# Autodesk Inventor assembly: RobotArm VersaPlanetaryGearbox
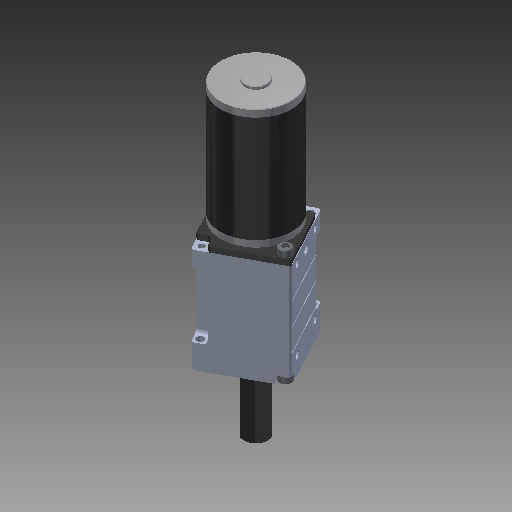
[picture p0: Inventor's stored thumbnail of the model, 512x512]
Saved by Autodesk Inventor 2018 (Build 220112000, 112)
## iProperties
Created: 2014-02-17
Part Number: RobotArm VersaPlanetaryGearbox
Description: STEP AP214
Document SubType Name: Assembly
Designer: lopez.xavier
Sending System: SolidWorks 2013
Preprocessor: SwSTEP 2.0
Title: BAG 2 stage Release.STEP
Author: IFMI-VEX04
Revision Number: ANY
## Documents named in this file (17)
- \\fs1\studentusers\class19\Lopez.Xavier\documents\RobotArm VersaPlanetaryGearbox.iam
- C:\Users\lopez.xavier.NICHOLSNT.000\Downloads\217-2625-001 Rev1.ipt
- C:\Users\lopez.xavier.NICHOLSNT.000\Downloads\217-2625-002 Rev1.ipt
- C:\Users\lopez.xavier.NICHOLSNT.000\Downloads\217-2625-003 Rev1.ipt
- C:\Users\lopez.xavier.NICHOLSNT.000\Downloads\217-2625-009 Rev1.ipt
- C:\Users\lopez.xavier.NICHOLSNT.000\Downloads\217-2625-100.iam
- C:\Users\lopez.xavier.NICHOLSNT.000\Downloads\217-2625-007 Rev1_Sun_Driver01.ipt
- C:\Users\lopez.xavier.NICHOLSNT.000\Downloads\217-2742.ipt
- C:\Users\lopez.xavier.NICHOLSNT.000\Downloads\SSS1032-0125ZB_94105A824.ipt
- C:\Users\lopez.xavier.NICHOLSNT.000\Downloads\217-3351.ipt
- C:\Users\lopez.xavier.NICHOLSNT.000\Downloads\217-2816-001 Rev1.ipt
- C:\Users\lopez.xavier.NICHOLSNT.000\Downloads\SSA_SSA0832-1750ZC.ipt
- C:\Users\lopez.xavier.NICHOLSNT.000\Downloads\217-2625-011 Rev1.ipt
- C:\Users\lopez.xavier.NICHOLSNT.000\Downloads\SSA_SSA0832-0500ZC.ipt
- C:\Users\lopez.xavier.NICHOLSNT.000\Downloads\SSHCM004_SSHCM004070010C.ipt
- C:\Users\lopez.xavier.NICHOLSNT.000\Downloads\217-2818 Rev1.iam
- C:\Users\lopez.xavier.NICHOLSNT.000\Downloads\217-2822-003 Rev4.ipt
## Components (21 placed, 21 different names)
1. 217-2625-001 Rev1_1 — Mate:41, Flush:10, Flush:11, Mate:49, Flush:13, Mate:57
2. 217-2625-002 Rev1_2 — Mate:13, Mate:15, Mate:16, Mate:17, Mate:18, Mate:19, Flush:12, Mate:50
3. 217-2625-003 Rev1_3 — Mate:11, Mate:14
4. 217-2625-009 Rev1_4 — Mate:20, Flush:9, Mate:27, Mate:47, Mate:48, Flush:13
5. 217-2625-100_5 [sub-assembly] — Mate:33, Mate:44, Mate:45
6. 217-2625-007 Rev1_Sun_Driver01_6 — Mate:47
7. 217-2742_7 — Mate:11, Mate:12, Mate:13, Mate:14, Mate:15
8. 217-2742_8 — Mate:12, Flush:12
9. SSS1032-0125ZB_94105A824_12 — Mate:27, Mate:46
10. 217-3351_14 — Mate:22, Mate:40, Mate:58
11. 217-2816-001 Rev1_15 — Mate:42, Mate:43, Mate:50, Mate:51, Mate:52
12. SSA_SSA0832-1750ZC_16 — Mate:16, Mate:17, Mate:54, Mate:56
13. SSA_SSA0832-1750ZC_17 — Mate:18, Mate:19, Mate:53, Mate:55
14. 217-2625-011 Rev1_18 — Mate:20, Flush:9, Mate:46
15. SSA_SSA0832-0500ZC_19 — Mate:37, Mate:39, Mate:55
16. SSA_SSA0832-0500ZC_20 — Mate:36, Mate:38, Mate:56
17. SSHCM004_SSHCM004070010C_21 — Mate:24, Mate:25
18. SSHCM004_SSHCM004070010C_22 — Mate:23, Mate:26, Mate:40
19. 217-2816-001 Rev1_23 — Mate:44, Mate:45, Mate:48, Mate:49, Mate:51, Mate:52, Mate:53, Mate:54, Mate:57
20. 217-2818 Rev1_24 [sub-assembly] — Mate:33, Mate:42, Mate:43
21. 217-2822-003 Rev4_25 — Mate:22, Mate:23, Mate:24, Mate:25, Mate:26, Mate:36, Mate:37, Mate:38, Mate:39, Mate:41, Flush:10, Flush:11, Mate:58
## Relationships (45: Mate 40, Flush 5)
- Mate:11: 217-2625-003 Rev1_3 ↔ 217-2742_7
- Mate:12: 217-2742_7 ↔ 217-2742_8
- Mate:13: 217-2625-002 Rev1_2 ↔ 217-2742_7
- Mate:14: 217-2625-003 Rev1_3 ↔ 217-2742_7
- Mate:15: 217-2625-002 Rev1_2 ↔ 217-2742_7
- Mate:16: 217-2625-002 Rev1_2 ↔ SSA_SSA0832-1750ZC_16
- Mate:17: 217-2625-002 Rev1_2 ↔ SSA_SSA0832-1750ZC_16
- Mate:18: 217-2625-002 Rev1_2 ↔ SSA_SSA0832-1750ZC_17
- Mate:19: 217-2625-002 Rev1_2 ↔ SSA_SSA0832-1750ZC_17
- Mate:20: 217-2625-009 Rev1_4 ↔ 217-2625-011 Rev1_18
- Flush:9: 217-2625-009 Rev1_4 ↔ 217-2625-011 Rev1_18
- Mate:22: 217-3351_14 ↔ 217-2822-003 Rev4_25
- Mate:23: SSHCM004_SSHCM004070010C_22 ↔ 217-2822-003 Rev4_25
- Mate:24: SSHCM004_SSHCM004070010C_21 ↔ 217-2822-003 Rev4_25
- Mate:25: SSHCM004_SSHCM004070010C_21 ↔ 217-2822-003 Rev4_25
- Mate:26: SSHCM004_SSHCM004070010C_22 ↔ 217-2822-003 Rev4_25
- Mate:27: 217-2625-009 Rev1_4 ↔ SSS1032-0125ZB_94105A824_12
- Mate:33: 217-2625-100_5 ↔ 217-2818 Rev1_24
- Mate:36: SSA_SSA0832-0500ZC_20 ↔ 217-2822-003 Rev4_25
- Mate:37: SSA_SSA0832-0500ZC_19 ↔ 217-2822-003 Rev4_25
- Mate:38: SSA_SSA0832-0500ZC_20 ↔ 217-2822-003 Rev4_25
- Mate:39: SSA_SSA0832-0500ZC_19 ↔ 217-2822-003 Rev4_25
- Mate:40: 217-3351_14 ↔ SSHCM004_SSHCM004070010C_22
- Mate:41: 217-2625-001 Rev1_1 ↔ 217-2822-003 Rev4_25
- Flush:10: 217-2625-001 Rev1_1 ↔ 217-2822-003 Rev4_25
- Flush:11: 217-2625-001 Rev1_1 ↔ 217-2822-003 Rev4_25
- Flush:12: 217-2625-002 Rev1_2 ↔ 217-2742_8
- Mate:42: 217-2816-001 Rev1_15 ↔ 217-2818 Rev1_24
- Mate:43: 217-2816-001 Rev1_15 ↔ 217-2818 Rev1_24
- Mate:44: 217-2625-100_5 ↔ 217-2816-001 Rev1_23
- Mate:45: 217-2625-100_5 ↔ 217-2816-001 Rev1_23
- Mate:46 (5.08 mm): SSS1032-0125ZB_94105A824_12 ↔ 217-2625-011 Rev1_18
- Mate:47: 217-2625-009 Rev1_4 ↔ 217-2625-007 Rev1_Sun_Driver01_6
- Mate:48: 217-2625-009 Rev1_4 ↔ 217-2816-001 Rev1_23
- Mate:49: 217-2625-001 Rev1_1 ↔ 217-2816-001 Rev1_23
- Mate:50: 217-2625-002 Rev1_2 ↔ 217-2816-001 Rev1_15
- Mate:51: 217-2816-001 Rev1_15 ↔ 217-2816-001 Rev1_23
- Mate:52: 217-2816-001 Rev1_15 ↔ 217-2816-001 Rev1_23
- Mate:53: SSA_SSA0832-1750ZC_17 ↔ 217-2816-001 Rev1_23
- Mate:54: SSA_SSA0832-1750ZC_16 ↔ 217-2816-001 Rev1_23
- Mate:55: SSA_SSA0832-1750ZC_17 ↔ SSA_SSA0832-0500ZC_19
- Mate:56: SSA_SSA0832-1750ZC_16 ↔ SSA_SSA0832-0500ZC_20
- Flush:13: 217-2625-001 Rev1_1 ↔ 217-2625-009 Rev1_4
- Mate:57: 217-2625-001 Rev1_1 ↔ 217-2816-001 Rev1_23
- Mate:58: 217-3351_14 ↔ 217-2822-003 Rev4_25
